# Autodesk Inventor assembly: Wide Assembly
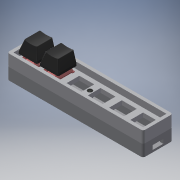
[picture p0: Inventor's stored thumbnail of the model, 180x180]
Saved by Autodesk Inventor 2018 (Build 220112000, 112)
## iProperties
Created: 2018-05-25
Part Number: Wide Assembly
Document SubType Name: Assembly
Designer: mtsti
Author: mtsti
## Documents named in this file (6)
- C:\Users\mtsti\Desktop\Macro Deck\Wide Assembly.iam
- C:\Users\mtsti\Desktop\Macro Deck\Base Wide.ipt
- C:\Users\mtsti\Desktop\Macro Deck\Key Plate Wide.ipt
- C:\Users\mtsti\Desktop\Macro Deck\Switch\cherry old.ipt
- C:\Users\mtsti\Desktop\Macro Deck\Keycap\MX 轴标准键帽.ipt
- C:\Users\mtsti\Desktop\Macro Deck\M2 Screw.ipt
## Components (7 placed, 5 different names)
1. Base Wide:1 — Flush:1, Flush:2, Mate:1
2. Key Plate Wide:1 — Flush:1, Flush:2, Mate:1, Mate:2, Mate:3, Mate:4, Mate:5, Mate:6, Mate:7, Mate:14, Mate:15
3. cherry old:1 — Mate:2, Mate:3, Mate:7, Mate:8, Mate:9, Mate:10
4. cherry old:2 — Mate:4, Mate:5, Mate:6, Mate:11, Mate:12, Mate:13
5. MX 轴标准键帽:1 — Mate:8, Mate:9, Mate:10
6. MX 轴标准键帽:2 — Mate:11, Mate:12, Mate:13
7. M2 Screw:1 — Mate:14, Mate:15
## Relationships (17: Mate 15, Flush 2)
- Flush:1: Base Wide:1 ↔ Key Plate Wide:1
- Flush:2: Base Wide:1 ↔ Key Plate Wide:1
- Mate:1: Base Wide:1 ↔ Key Plate Wide:1
- Mate:2: Key Plate Wide:1 ↔ cherry old:1
- Mate:3: Key Plate Wide:1 ↔ cherry old:1
- Mate:4: Key Plate Wide:1 ↔ cherry old:2
- Mate:5: Key Plate Wide:1 ↔ cherry old:2
- Mate:6: Key Plate Wide:1 ↔ cherry old:2
- Mate:7: Key Plate Wide:1 ↔ cherry old:1
- Mate:8: cherry old:1 ↔ MX 轴标准键帽:1
- Mate:9: cherry old:1 ↔ MX 轴标准键帽:1
- Mate:10: cherry old:1 ↔ MX 轴标准键帽:1
- Mate:11: cherry old:2 ↔ MX 轴标准键帽:2
- Mate:12: cherry old:2 ↔ MX 轴标准键帽:2
- Mate:13: cherry old:2 ↔ MX 轴标准键帽:2
- Mate:14: Key Plate Wide:1 ↔ M2 Screw:1
- Mate:15: Key Plate Wide:1 ↔ M2 Screw:1
